# Autodesk Inventor assembly: ASY GBK 3110 wall shield Center 1
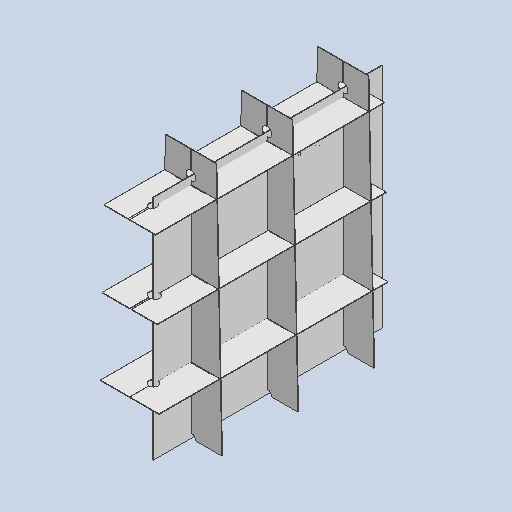
[picture p0: Inventor's stored thumbnail of the model, 512x512]
Saved by Autodesk Inventor 2026 (Build 300175000, 175)
## iProperties
Created: 2026-05-19
Part Number: ASY GBK 3110 wall shield Center 1
Document SubType Name: Assembly
Designer: admin
Mass: 174041 g
Surface Area: 113034 cm^2
Volume: 22170.8 cm^3
Density: 7.85 g/cm^3
Author: admin
## Documents named in this file (6)
- C:\Users\pokla\Documents\Inventor\GBK-Gubkinskiy\ASY GBK 3110 wall shield Center 1.iam
- C:\Users\pokla\Documents\Inventor\GBK-Gubkinskiy\GBK 3101 Center main rib.ipt
- C:\Users\pokla\Documents\Inventor\GBK-Gubkinskiy\GBK 3102 stringer 1.ipt
- C:\Users\pokla\Documents\Inventor\GBK-Gubkinskiy\GBK 1111 shield 1.ipt
- C:\Users\pokla\Documents\Inventor\GBK-Gubkinskiy\GBK 3103 stringer 2.ipt
- C:\Users\pokla\Documents\Inventor\GBK-Gubkinskiy\GBK 3104 stringer 3.ipt
## Components (13 placed, 5 different names)
1. GBK 3102 stringer 1.ipt:1 — Жесткий:1
2. GBK 1111 shield 1.ipt:1 — Совмещение:1, Заподлицо:1, Совмещение:2, Заподлицо:2, Совмещение:4, Заподлицо:3, Совмещение:5, Заподлицо:5
3. GBK 3103 stringer 2.ipt:1 — Жесткий:2
4. GBK 3104 stringer 3.ipt:1 — Жесткий:3
5. GBK 3102 stringer 1.ipt:2 — Жесткий:6
6. GBK 3103 stringer 2.ipt:2 — Жесткий:5
7. GBK 3104 stringer 3.ipt:2 — Жесткий:4
8. GBK 3101 Center main rib.ipt:1 — Жесткий:1, Заподлицо:3, Совмещение:5, Заподлицо:4, Заподлицо:5, Жесткий:2, Жесткий:3
9. GBK 3101 Center main rib.ipt:2 — Заподлицо:2, Совмещение:4, Заподлицо:4, Жесткий:4, Жесткий:5, Жесткий:6
10. GBK 3101 Center main rib.ipt:3
11. GBK 3101 Center main rib.ipt:4
12. GBK 3101 Center main rib.ipt:5
13. GBK 3101 Center main rib.ipt:6
## Component patterns: (3 elements, first: GBK 3101 Center main rib.ipt:1 + GBK 3101 Center main rib.ipt:2)
## Relationships (15: WeldJoint 6, Flush 5, Mate 4)
- Жесткий:1 [WeldJoint] (4 mm): GBK 3102 stringer 1.ipt:1 ↔ GBK 3101 Center main rib.ipt:1
- Совмещение:1 [Mate]: GBK 1111 shield 1.ipt:1
- Заподлицо:1 [Flush]: GBK 1111 shield 1.ipt:1
- Совмещение:2 [Mate]: GBK 1111 shield 1.ipt:1
- Заподлицо:2 [Flush]: GBK 1111 shield 1.ipt:1 ↔ GBK 3101 Center main rib.ipt:2
- Совмещение:4 [Mate]: GBK 1111 shield 1.ipt:1 ↔ GBK 3101 Center main rib.ipt:2
- Заподлицо:3 [Flush]: GBK 1111 shield 1.ipt:1 ↔ GBK 3101 Center main rib.ipt:1
- Совмещение:5 [Mate]: GBK 1111 shield 1.ipt:1 ↔ GBK 3101 Center main rib.ipt:1
- Заподлицо:4 [Flush]: GBK 3101 Center main rib.ipt:1 ↔ GBK 3101 Center main rib.ipt:2
- Заподлицо:5 [Flush] (250 mm): GBK 1111 shield 1.ipt:1 ↔ GBK 3101 Center main rib.ipt:1
- Жесткий:2 [WeldJoint] (4 mm): GBK 3103 stringer 2.ipt:1 ↔ GBK 3101 Center main rib.ipt:1
- Жесткий:3 [WeldJoint] (4 mm): GBK 3104 stringer 3.ipt:1 ↔ GBK 3101 Center main rib.ipt:1
- Жесткий:4 [WeldJoint]: GBK 3104 stringer 3.ipt:2 ↔ GBK 3101 Center main rib.ipt:2
- Жесткий:5 [WeldJoint]: GBK 3103 stringer 2.ipt:2 ↔ GBK 3101 Center main rib.ipt:2
- Жесткий:6 [WeldJoint]: GBK 3102 stringer 1.ipt:2 ↔ GBK 3101 Center main rib.ipt:2
